# Autodesk Inventor assembly: Phone assembly solution
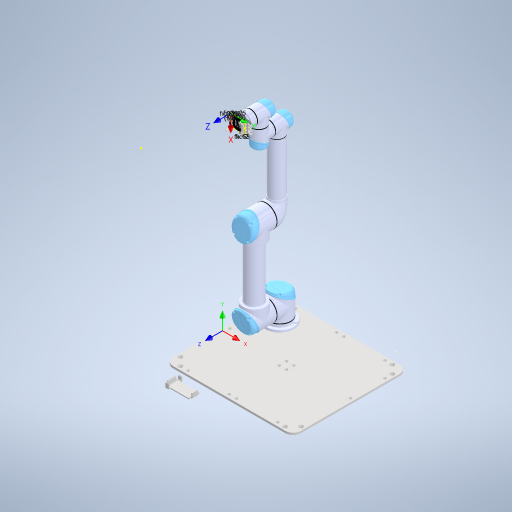
[picture p0: Inventor's stored thumbnail of the model, 512x512]
Saved by Autodesk Inventor 2024 (Build 280153000, 153)
## iProperties
Created: 2024-03-26
Part Number: Phone assembly solution
Document SubType Name: Assembly
Designer: jens1
Author: jens1
## Documents named in this file (12)
- C:\Users\jens1\Documents\GitHub\Robotteknologi-2.-semester\3D modeller\Phone assembly solution.iam
- C:\Users\jens1\Documents\GitHub\Robotteknologi-2.-semester\3D modeller\UR5\UR5\UR5.iam
- C:\Users\jens1\Documents\GitHub\Robotteknologi-2.-semester\3D modeller\Mount plate UR.ipt
- C:\Users\jens1\Documents\GitHub\Robotteknologi-2.-semester\3D modeller\Left bottom plate.ipt
- C:\Users\jens1\Documents\GitHub\Robotteknologi-2.-semester\3D modeller\Right bottom plate.ipt
- C:\Users\jens1\Documents\GitHub\Robotteknologi-2.-semester\3D modeller\Right top plate.ipt
- C:\Users\jens1\Documents\GitHub\Robotteknologi-2.-semester\3D modeller\Phone\Sikring.ipt
- C:\Users\jens1\Documents\GitHub\Robotteknologi-2.-semester\3D modeller\Gripper\Gripper.iam
- C:\Users\jens1\Documents\GitHub\Robotteknologi-2.-semester\3D modeller\Phone\Bund.ipt
- C:\Users\jens1\Documents\GitHub\Robotteknologi-2.-semester\3D modeller\Phone\Top.ipt
- C:\Users\jens1\Documents\GitHub\Robotteknologi-2.-semester\3D modeller\Phone\PCB.ipt
- C:\Users\jens1\Documents\GitHub\Robotteknologi-2.-semester\3D modeller\Mounting station.ipt
## Components (11 placed, 11 different names)
1. UR5:1 [sub-assembly] — Mate:2, Mate:3, Mate:4, Tangent:1, Mate:9, Mate:10, Mate:11
2. Mount plate UR:1 — Mate:1, Mate:2, Mate:3, Mate:4, Tangent:1, Flush:1, Mate:5, Flush:2, Flush:5, Mate:8
3. Left bottom plate:1 — Flush:1, Mate:5, Flush:2, Flush:3, Mate:6, Flush:4
4. Right bottom plate:1 — Flush:3, Mate:6, Flush:4, Mate:7
5. Right top plate:1 — Flush:5, Mate:7, Mate:8
6. Gripper:1 [sub-assembly] — Mate:9, Mate:10, Mate:11
7. Sikring:2
8. Bund:1
9. Top:1 — Mate:12, Tangent:2, Flush:6
10. PCB:1 — Mate:12, Tangent:2, Flush:6
11. Mounting station:1
## Relationships (20: Mate 12, Flush 6, Tangent 2)
- Mate:1: Mount plate UR:1
- Mate:2: UR5:1 ↔ Mount plate UR:1
- Mate:3 (-116 mm): UR5:1 ↔ Mount plate UR:1
- Mate:4 (-116 mm): UR5:1 ↔ Mount plate UR:1
- Tangent:1 (0.25 mm): UR5:1 ↔ Mount plate UR:1
- Flush:1: Mount plate UR:1 ↔ Left bottom plate:1
- Mate:5: Mount plate UR:1 ↔ Left bottom plate:1
- Flush:2: Mount plate UR:1 ↔ Left bottom plate:1
- Flush:3: Left bottom plate:1 ↔ Right bottom plate:1
- Mate:6: Left bottom plate:1 ↔ Right bottom plate:1
- Flush:4: Left bottom plate:1 ↔ Right bottom plate:1
- Flush:5: Mount plate UR:1 ↔ Right top plate:1
- Mate:7: Right bottom plate:1 ↔ Right top plate:1
- Mate:8: Mount plate UR:1 ↔ Right top plate:1
- Mate:9: UR5:1 ↔ Gripper:1
- Mate:10: UR5:1 ↔ Gripper:1
- Mate:11: UR5:1 ↔ Gripper:1
- Mate:12: Top:1 ↔ PCB:1
- Tangent:2 (3.5 mm): Top:1 ↔ PCB:1
- Flush:6 (18.25 mm): Top:1 ↔ PCB:1
